# Autodesk Inventor assembly: Palma
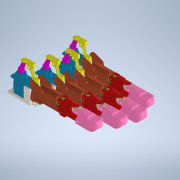
[picture p0: Inventor's stored thumbnail of the model, 180x180]
Saved by Autodesk Inventor 2020 (Build 240168000, 168)
## iProperties
Created: 2021-08-20
Part Number: Palma
Document SubType Name: Assembly
Designer: chalo
Author: chalo
## Documents named in this file (2)
- C:\Users\chalo\OneDrive\Documents\GitHub\Interfaces-Biomedicas-2021\Gonzalo Palarea\Inventor\_completa\Palma.iam
- C:\Users\chalo\OneDrive\Documents\GitHub\Interfaces-Biomedicas-2021\Gonzalo Palarea\Inventor\tipo2\Prototipo2.iam
## Components (4 placed, 1 different names)
1. Prototipo2:1 [sub-assembly] — Flush:1, Flush:2, Flush:3, Mate:1, Flush:4
2. Prototipo2:2 [sub-assembly] — Flush:1, Mate:1, Mate:2, Flush:4, Flush:5
3. Prototipo2:3 [sub-assembly] — Flush:2, Mate:2, Mate:3, Flush:5, Flush:6
4. Prototipo2:4 [sub-assembly] — Flush:3, Mate:3, Flush:6
## Relationships (9: Flush 6, Mate 3)
- Flush:1: Prototipo2:1 ↔ Prototipo2:2
- Flush:2: Prototipo2:1 ↔ Prototipo2:3
- Flush:3: Prototipo2:1 ↔ Prototipo2:4
- Mate:1 (7 mm): Prototipo2:1 ↔ Prototipo2:2
- Mate:2 (7 mm): Prototipo2:2 ↔ Prototipo2:3
- Mate:3 (7 mm): Prototipo2:3 ↔ Prototipo2:4
- Flush:4 (-15 mm): Prototipo2:1 ↔ Prototipo2:2
- Flush:5 (-7 mm): Prototipo2:2 ↔ Prototipo2:3
- Flush:6 (-12 mm): Prototipo2:3 ↔ Prototipo2:4
